# Autodesk Inventor assembly: Plastic Box with Batteries and Spacer
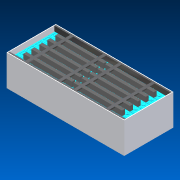
[picture p0: Inventor's stored thumbnail of the model, 180x180]
Saved by Autodesk Inventor 2012 (Build 160160000, 160)
## iProperties
Created: 2012-07-02
Part Number: Plastic Box with Batteries and Spacer
Document SubType Name: Assembly
Designer: Hemant
Author: Hemant
## Documents named in this file (6)
- C:\Users\Hemant\Documents\Battery Boxes\BB REAR A\Plastic Box with Batteries and Spacer.iam
- C:\Users\Hemant\Documents\Battery Boxes\BB REAR A\Plastic Box\Plstic Box Rear A Assembly.iam
- C:\Users\Hemant\Documents\Battery Boxes\Batteries\REAR A Battery Pack.iam
- C:\Users\Hemant\Documents\Battery Boxes\BB REAR A\spacer 2.ipt
- C:\Users\Hemant\Documents\Battery Boxes\BB REAR A\mid spacer.ipt
- C:\Users\Hemant\Documents\Battery Boxes\BB REAR A\spacer 3.ipt
## Components (18 placed, 5 different names)
1. REAR A Battery Pack:1 [sub-assembly] — Mate:22, Mate:25, Mate:26, Mate:30, Mate:32, Mate:36
2. Plstic Box Rear A Assembly:1 [sub-assembly] — Mate:22, Mate:25, Mate:26, Mate:29, Mate:31, Mate:33, Mate:34, Mate:39, Mate:40, Mate:41
3. spacer 2:1 — Mate:29, Mate:30, Mate:31, Mate:37, Flush:3
4. spacer 2:2 — Mate:32, Mate:33, Mate:34
5. mid spacer:1 — Flush:2, Mate:42
6. mid spacer:2
7. mid spacer:3
8. mid spacer:4 — Mate:36
9. mid spacer:5 — Mate:35, Flush:1
10. mid spacer:6 — Flush:2, Mate:38
11. mid spacer:8
12. mid spacer:9
13. mid spacer:10
14. mid spacer:11 — Mate:35, Flush:1, Mate:37, Flush:3
15. spacer 3:1 — Flush:4
16. spacer 3:2 — Mate:38, Mate:39, Mate:40
17. spacer 3:3 — Flush:4, Mate:41, Mate:42
18. spacer 3:4
## Component patterns: (5 elements, first: mid spacer:1), (5 elements, first: mid spacer:6), (2 elements, first: spacer 3:1), (2 elements, first: spacer 3:3)
## Relationships (21: Mate 17, Flush 4)
- Mate:22: REAR A Battery Pack:1 ↔ Plstic Box Rear A Assembly:1
- Mate:25 (1.4224 mm): REAR A Battery Pack:1 ↔ Plstic Box Rear A Assembly:1
- Mate:26 (3.9116 mm): REAR A Battery Pack:1 ↔ Plstic Box Rear A Assembly:1
- Mate:29: Plstic Box Rear A Assembly:1 ↔ spacer 2:1
- Mate:30: REAR A Battery Pack:1 ↔ spacer 2:1
- Mate:31: Plstic Box Rear A Assembly:1 ↔ spacer 2:1
- Mate:32: REAR A Battery Pack:1 ↔ spacer 2:2
- Mate:33: Plstic Box Rear A Assembly:1 ↔ spacer 2:2
- Mate:34: Plstic Box Rear A Assembly:1 ↔ spacer 2:2
- Mate:35 (12.7 mm): mid spacer:5 ↔ mid spacer:11
- Flush:1: mid spacer:5 ↔ mid spacer:11
- Flush:2: mid spacer:1 ↔ mid spacer:6
- Mate:36: REAR A Battery Pack:1 ↔ mid spacer:4
- Mate:37 (43.18 mm): spacer 2:1 ↔ mid spacer:11
- Flush:3: spacer 2:1 ↔ mid spacer:11
- Mate:38: mid spacer:6 ↔ spacer 3:2
- Mate:39: Plstic Box Rear A Assembly:1 ↔ spacer 3:2
- Mate:40: Plstic Box Rear A Assembly:1 ↔ spacer 3:2
- Flush:4: spacer 3:1 ↔ spacer 3:3
- Mate:41: Plstic Box Rear A Assembly:1 ↔ spacer 3:3
- Mate:42: mid spacer:1 ↔ spacer 3:3
